# Autodesk Inventor assembly: Placa_generica
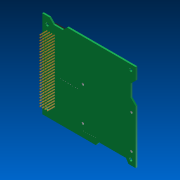
[picture p0: Inventor's stored thumbnail of the model, 180x180]
Saved by Autodesk Inventor 2012 (Build 160160000, 160)
## iProperties
Created: 2016-01-12
Part Number: Placa_generica
Document SubType Name: Assembly
Designer: Alex Becerra
Mass: 50.3 g
Surface Area: 251.917 cm^2
Volume: 18.9436 cm^3
Density: 2.65525 g/cm^3
Author: Alex Becerra
## Documents named in this file (3)
- C:\Users\Thinkpad\Cubesat SUChAI\Mecanica\Modelo_3D\Anexos\Placa_generica.iam
- C:\Users\Thinkpad\Cubesat SUChAI\Mecanica\Modelo_3D\Placa_payloads\Placa_base\placa_pc104.ipt
- C:\Users\Thinkpad\Cubesat SUChAI\Mecanica\Modelo_3D\Conectores_y_separadores\esq-102-03-g-d.ipt
## Components (2 placed, 2 different names)
1. placa_pc104:1 — Mate:1, Mate:2, Mate:3
2. esq-102-03-g-d:1 — Mate:1, Mate:2, Mate:3
## Relationships (3: Mate 3)
- Mate:1: placa_pc104:1 ↔ esq-102-03-g-d:1
- Mate:2: placa_pc104:1 ↔ esq-102-03-g-d:1
- Mate:3: placa_pc104:1 ↔ esq-102-03-g-d:1
